# Autodesk Inventor assembly: Baterías
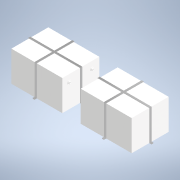
[picture p0: Inventor's stored thumbnail of the model, 180x180]
Saved by Autodesk Inventor 2022.1 (Build 261234000, 234)
## iProperties
Created: 2021-10-01
Part Number: Baterías
Document SubType Name: Assembly
Designer: seb_0
Mass: 33006.4 g
Surface Area: 8204.7 cm^2
Volume: 18507.6 cm^3
Density: 1.7834 g/cm^3
Author: seb_0
## Documents named in this file (3)
- C:\Users\seb_0\Desktop\PDM\ProyectoRobotPallet\Batería\Baterías.iam
- C:\Users\seb_0\Desktop\PDM\ProyectoRobotPallet\Batería\Batería.ipt
- C:\Users\seb_0\Desktop\PDM\ProyectoRobotPallet\Batería\Soporte.ipt
## Components (4 placed, 2 different names)
1. Batería:1 — Coincidencia:1, Coincidencia:2, Nivelación:1, Coincidencia:3, Nivelación:2, Nivelación:4, Coincidencia:6, Coincidencia:7
2. Batería:2 — Nivelación:1, Coincidencia:3, Nivelación:2, Coincidencia:4, Coincidencia:5, Nivelación:3
3. Soporte:1 — Coincidencia:4, Coincidencia:5, Nivelación:3
4. Soporte:2 — Nivelación:4, Coincidencia:6, Coincidencia:7
## Relationships (11: Mate 7, Flush 4)
- Coincidencia:1 [Mate]: Batería:1
- Coincidencia:2 [Mate]: Batería:1
- Nivelación:1 [Flush]: Batería:1 ↔ Batería:2
- Coincidencia:3 [Mate] (100 mm): Batería:1 ↔ Batería:2
- Nivelación:2 [Flush]: Batería:1 ↔ Batería:2
- Coincidencia:4 [Mate]: Batería:2 ↔ Soporte:1
- Coincidencia:5 [Mate]: Batería:2 ↔ Soporte:1
- Nivelación:3 [Flush]: Batería:2 ↔ Soporte:1
- Nivelación:4 [Flush]: Batería:1 ↔ Soporte:2
- Coincidencia:6 [Mate]: Batería:1 ↔ Soporte:2
- Coincidencia:7 [Mate]: Batería:1 ↔ Soporte:2
